# Autodesk Inventor assembly: 足回り_MIR
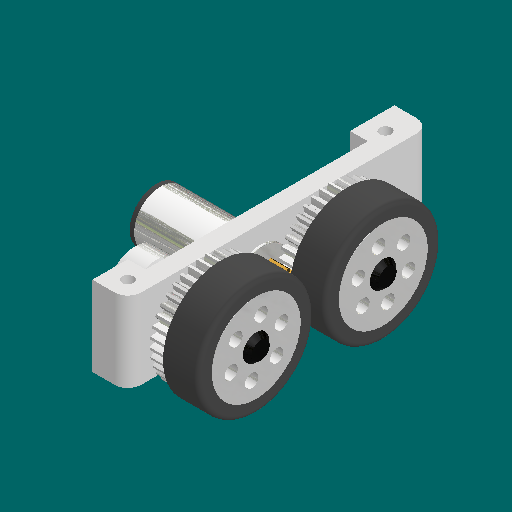
[picture p0: Inventor's stored thumbnail of the model, 512x512]
Saved by Autodesk Inventor 2023 (Build 270158000, 158)
## iProperties
Created: 2022-03-31
Part Number: 足回り_MIR
Document SubType Name: Assembly
Designer: hide
Author: neko2
## Documents named in this file (12)
- C:\Users\hide\Desktop\SaponseEx\CAD\mirror\足回り_MIR.iam
- C:\Users\hide\Desktop\SaponseEx\CAD\mirror\CoreLessMotor_MIR.ipt
- C:\Users\hide\Desktop\SaponseEx\CAD\mirror\FL673ZZ_MIR.ipt
- C:\Users\hide\Desktop\SaponseEx\CAD\mirror\HeikoPin_MIR.ipt
- C:\Users\hide\Desktop\SaponseEx\CAD\mirror\RT-PN v2_MIR.ipt
- C:\Users\hide\Desktop\SaponseEx\CAD\mirror\Tire_MIR.ipt
- C:\Users\hide\Desktop\SaponseEx\CAD\mirror\Stopper_MIR.ipt
- C:\Users\hide\Desktop\SaponseEx\CAD\mirror\Magnet_MIR.iam
- C:\Users\hide\Desktop\SaponseEx\CAD\mirror\Magnet_Simple_MIR.ipt
- C:\Users\hide\Desktop\SaponseEx\CAD\mirror\Magnet_MIR.ipt
- C:\Users\hide\Desktop\SaponseEx\CAD\mirror\Gear_MIR.iam
- C:\Users\hide\Desktop\SaponseEx\CAD\mirror\MotorMount_New_MIR.ipt
## Components (17 placed, 10 different names)
1. CoreLessMotor_MIR:1 — 回転:1, リジッド:31
2. FL673ZZ_MIR:1 — メイト:29, リジッド:33
3. FL673ZZ_MIR:2 — メイト:36, 円柱状:22, リジッド:34
4. FL673ZZ_MIR:3 — メイト:37, リジッド:35
5. FL673ZZ_MIR:4 — メイト:32, 円柱状:21, リジッド:32
6. HeikoPin_MIR:1 — 円柱状:22, 円柱状:17, 円柱状:19, リジッド:28
7. HeikoPin_MIR:2 — メイト:38, 円柱状:21, 円柱状:18, 円柱状:20
8. RT-PN v2_MIR:1 — 回転:1
9. Tire_MIR:1 — リジッド:30
10. Tire_MIR:2 — リジッド:29
11. Stopper_MIR:1 — メイト:29, 円柱状:18
12. Magnet_MIR:1 [sub-assembly] — 円柱状:17
13. Magnet_Simple_MIR:1 — メイト:37, 円柱状:19, リジッド:27
14. Magnet_MIR:2 — リジッド:27
15. Gear_MIR:1 [sub-assembly] — メイト:38, メイト:32, リジッド:30, 円柱状:20
16. Gear_MIR:2 [sub-assembly] — メイト:36, リジッド:29, リジッド:28
17. MotorMount_New_MIR:1 — メイト:35, フラッシュ:36, メイト:34, リジッド:35, リジッド:34, リジッド:33, リジッド:32, リジッド:31
## Relationships (24: WeldJoint 9, Mate 7, CylindricalJoint 6, Flush 1, RevoluteJoint 1)
- メイト:29 [Mate]: FL673ZZ_MIR:1 ↔ Stopper_MIR:1
- メイト:37 [Mate]: FL673ZZ_MIR:3 ↔ Magnet_Simple_MIR:1
- メイト:38 [Mate]: HeikoPin_MIR:2 ↔ Gear_MIR:1
- メイト:32 [Mate]: FL673ZZ_MIR:4 ↔ Gear_MIR:1
- メイト:36 [Mate]: FL673ZZ_MIR:2 ↔ Gear_MIR:2
- メイト:35 [Mate]: MotorMount_New_MIR:1
- フラッシュ:36 [Flush]: MotorMount_New_MIR:1
- メイト:34 [Mate]: MotorMount_New_MIR:1
- 円柱状:22 [CylindricalJoint]: FL673ZZ_MIR:2 ↔ HeikoPin_MIR:1
- 円柱状:21 [CylindricalJoint]: FL673ZZ_MIR:4 ↔ HeikoPin_MIR:2
- 円柱状:18 [CylindricalJoint]: HeikoPin_MIR:2 ↔ Stopper_MIR:1
- 円柱状:17 [CylindricalJoint]: HeikoPin_MIR:1 ↔ Magnet_MIR:1
- 円柱状:19 [CylindricalJoint]: HeikoPin_MIR:1 ↔ Magnet_Simple_MIR:1
- リジッド:27 [WeldJoint]: Magnet_Simple_MIR:1 ↔ Magnet_MIR:2
- リジッド:30 [WeldJoint]: Tire_MIR:1 ↔ Gear_MIR:1
- 円柱状:20 [CylindricalJoint]: HeikoPin_MIR:2 ↔ Gear_MIR:1
- リジッド:29 [WeldJoint]: Tire_MIR:2 ↔ Gear_MIR:2
- リジッド:28 [WeldJoint]: HeikoPin_MIR:1 ↔ Gear_MIR:2
- 回転:1 [RevoluteJoint] (-0.2 mm): CoreLessMotor_MIR:1 ↔ RT-PN v2_MIR:1
- リジッド:35 [WeldJoint]: FL673ZZ_MIR:3 ↔ MotorMount_New_MIR:1
- リジッド:34 [WeldJoint]: FL673ZZ_MIR:2 ↔ MotorMount_New_MIR:1
- リジッド:33 [WeldJoint]: FL673ZZ_MIR:1 ↔ MotorMount_New_MIR:1
- リジッド:32 [WeldJoint]: FL673ZZ_MIR:4 ↔ MotorMount_New_MIR:1
- リジッド:31 [WeldJoint]: CoreLessMotor_MIR:1 ↔ MotorMount_New_MIR:1
